# Autodesk Inventor assembly: 車輪パーツ
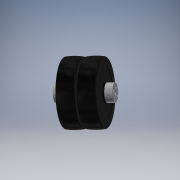
[picture p0: Inventor's stored thumbnail of the model, 180x180]
Saved by Autodesk Inventor 2019 (Build 230136000, 136)
## iProperties
Created: 2020-10-22
Part Number: 車輪パーツ
Material: 一般
Document SubType Name: Assembly
Designer: zhept
Author: zhept
## Documents named in this file (3)
- C:\Users\zhept\OneDrive\大学\rrst\足回り2020\車輪パーツ.iam
- C:\Users\zhept\OneDrive\大学\rrst\足回り2020\足回り試作2020_v1\HAMMER_CASTER_425ER100.ipt
- C:\Users\zhept\OneDrive\大学\rrst\足回り2020\足回り試作2020_v1\SCS0812CP3.iam
## Components (4 placed, 2 different names)
1. HAMMER_CASTER_425ER100:1
2. HAMMER_CASTER_425ER100:2
3. SCS0812CP3:1 [sub-assembly]
4. SCS0812CP3:2 [sub-assembly]
## Relationships (4: Mate 3, Angle 1)
- [Mate]: HAMMER_CASTER_425ER100:1 ↔ HAMMER_CASTER_425ER100:2
- [Angle] (0 deg): HAMMER_CASTER_425ER100:1 ↔ HAMMER_CASTER_425ER100:2
- [Mate]: HAMMER_CASTER_425ER100:2 ↔ SCS0812CP3:2
- [Mate]: HAMMER_CASTER_425ER100:1 ↔ SCS0812CP3:1
## Named parameters: d48_d46 = 0 mm, d49_d47 = 0 deg
